# Autodesk Inventor assembly: Camera assembly
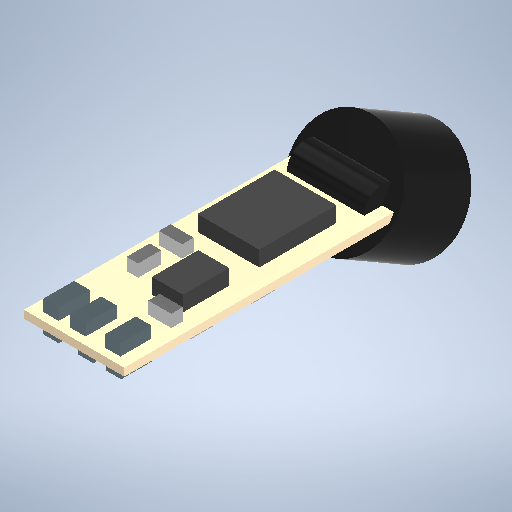
[picture p0: Inventor's stored thumbnail of the model, 512x512]
Saved by Autodesk Inventor 2026.2 (Build 302298010, 298A)
## iProperties
Created: 2026-04-26
Part Number: Camera assembly
Document SubType Name: Assembly
Designer: piete
Author: piete
## Documents named in this file (8)
- C:\Users\piete\Desktop\Skripsie\Documents\Detail Design\Micro Robotics Camera Module\Camera assembly.iam
- C:\Users\piete\Desktop\Skripsie\Documents\Detail Design\Micro Robotics Camera Module\PCB.ipt
- C:\Users\piete\Desktop\Skripsie\Documents\Detail Design\Micro Robotics Camera Module\Epoxy.ipt
- C:\Users\piete\Desktop\Skripsie\Documents\Detail Design\Micro Robotics Camera Module\Electrical Component.ipt
- C:\Users\piete\Desktop\Skripsie\Documents\Detail Design\Micro Robotics Camera Module\Camera and LED sensor.ipt
- C:\Users\piete\Desktop\Skripsie\Documents\Detail Design\Micro Robotics Camera Module\E Component 1.ipt
- C:\Users\piete\Desktop\Skripsie\Documents\Detail Design\Micro Robotics Camera Module\Resitors.ipt
- C:\Users\piete\Desktop\Skripsie\Documents\Detail Design\Micro Robotics Camera Module\Solder points.ipt
## Components (19 placed, 7 different names)
1. PCB:1 — Flush:1, Mate:1, Mate:2, Flush:2, Flush:3, Mate:3, Mate:5, Mate:6, Flush:4, Flush:5, Mate:7, Mate:8, Mate:9, Mate:10, Mate:15, Mate:16, Mate:17, Mate:18, Mate:19, Flush:8, Flush:9, Flush:10, Flush:11, Flush:12, Flush:13, Flush:14, Flush:15, Flush:16, Flush:17, Mate:20, Mate:21, Mate:22, Flush:18, Flush:19, Flush:20, Flush:21, Flush:22, Flush:23, Mate:23, Mate:24, Mate:25, Flush:24, Flush:25, Flush:26, Flush:27, Flush:28, Flush:29
2. Epoxy:1 — Flush:1, Mate:1, Mate:2, Mate:4
3. Electrical Component:1 — Flush:2, Flush:3, Mate:3, Mate:12, Flush:7
4. Camera and LED sensor:1 — Mate:4, Mate:5, Mate:6
5. E Component 1:1 — Flush:4, Flush:5, Mate:7, Mate:11, Flush:6, Mate:13
6. Resitors:1 — Mate:9, Mate:12, Flush:7, Mate:14
7. Resitors:2 — Mate:10, Mate:11, Flush:6
8. Resitors:3 — Mate:8, Mate:13, Mate:14
9. Resitors:4 — Mate:16, Flush:10, Flush:13
10. Resitors:5 — Mate:18, Flush:15, Flush:16
11. Resitors:6 — Mate:17, Flush:8, Flush:11
12. Resitors:7 — Mate:15, Flush:9, Flush:12
13. Resitors:8 — Mate:19, Flush:14, Flush:17
14. Solder points:1 — Mate:20, Flush:19, Flush:22
15. Solder points:2 — Mate:21, Flush:18, Flush:21
16. Solder points:3 — Mate:22, Flush:20, Flush:23
17. Solder points:4 — Mate:25, Flush:26, Flush:29
18. Solder points:5 — Mate:24, Flush:25, Flush:28
19. Solder points:6 — Mate:23, Flush:24, Flush:27
## Relationships (54: Flush 29, Mate 25)
- Flush:1 (-0.75 mm): PCB:1 ↔ Epoxy:1
- Mate:1: PCB:1 ↔ Epoxy:1
- Mate:2: PCB:1 ↔ Epoxy:1
- Flush:2 (1.25 mm): PCB:1 ↔ Electrical Component:1
- Flush:3 (2.5 mm): PCB:1 ↔ Electrical Component:1
- Mate:3: PCB:1 ↔ Electrical Component:1
- Mate:4: Epoxy:1 ↔ Camera and LED sensor:1
- Mate:5: PCB:1 ↔ Camera and LED sensor:1
- Mate:6: PCB:1 ↔ Camera and LED sensor:1
- Flush:4 (1.2 mm): PCB:1 ↔ E Component 1:1
- Flush:5 (5 mm): PCB:1 ↔ E Component 1:1
- Mate:7: PCB:1 ↔ E Component 1:1
- Mate:8: PCB:1 ↔ Resitors:3
- Mate:9: PCB:1 ↔ Resitors:1
- Mate:10: PCB:1 ↔ Resitors:2
- Mate:11 (0.5 mm): E Component 1:1 ↔ Resitors:2
- Flush:6 (-0.5 mm): E Component 1:1 ↔ Resitors:2
- Mate:12 (1.25 mm): Electrical Component:1 ↔ Resitors:1
- Flush:7 (-0.5 mm): Electrical Component:1 ↔ Resitors:1
- Mate:13 (1.4 mm): E Component 1:1 ↔ Resitors:3
- Mate:14 (1 mm): Resitors:1 ↔ Resitors:3
- Mate:15: PCB:1 ↔ Resitors:7
- Mate:16: PCB:1 ↔ Resitors:4
- Mate:17: PCB:1 ↔ Resitors:6
- Mate:18: PCB:1 ↔ Resitors:5
- Mate:19: PCB:1 ↔ Resitors:8
- Flush:8 (1 mm): PCB:1 ↔ Resitors:6
- Flush:9 (1 mm): PCB:1 ↔ Resitors:7
- Flush:10 (1 mm): PCB:1 ↔ Resitors:4
- Flush:11 (5 mm): PCB:1 ↔ Resitors:6
- Flush:12 (7.5 mm): PCB:1 ↔ Resitors:7
- Flush:13 (10 mm): PCB:1 ↔ Resitors:4
- Flush:14 (0.75 mm): PCB:1 ↔ Resitors:8
- Flush:15 (0.75 mm): PCB:1 ↔ Resitors:5
- Flush:16 (5 mm): PCB:1 ↔ Resitors:5
- Flush:17 (9 mm): PCB:1 ↔ Resitors:8
- Mate:20: PCB:1 ↔ Solder points:1
- Mate:21: PCB:1 ↔ Solder points:2
- Mate:22: PCB:1 ↔ Solder points:3
- Flush:18 (0.5 mm): PCB:1 ↔ Solder points:2
- Flush:19 (0.5 mm): PCB:1 ↔ Solder points:1
- Flush:20 (0.5 mm): PCB:1 ↔ Solder points:3
- Flush:21 (0.7 mm): PCB:1 ↔ Solder points:2
- Flush:22 (2.5 mm): PCB:1 ↔ Solder points:1
- Flush:23 (-0.75 mm): PCB:1 ↔ Solder points:3
- Mate:23: PCB:1 ↔ Solder points:6
- Mate:24: PCB:1 ↔ Solder points:5
- Mate:25: PCB:1 ↔ Solder points:4
- Flush:24 (0.5 mm): PCB:1 ↔ Solder points:6
- Flush:25 (0.5 mm): PCB:1 ↔ Solder points:5
- Flush:26 (0.5 mm): PCB:1 ↔ Solder points:4
- Flush:27 (0.75 mm): PCB:1 ↔ Solder points:6
- Flush:28 (2.5 mm): PCB:1 ↔ Solder points:5
- Flush:29 (0.75 mm): PCB:1 ↔ Solder points:4
